# Autodesk Inventor assembly: стенка
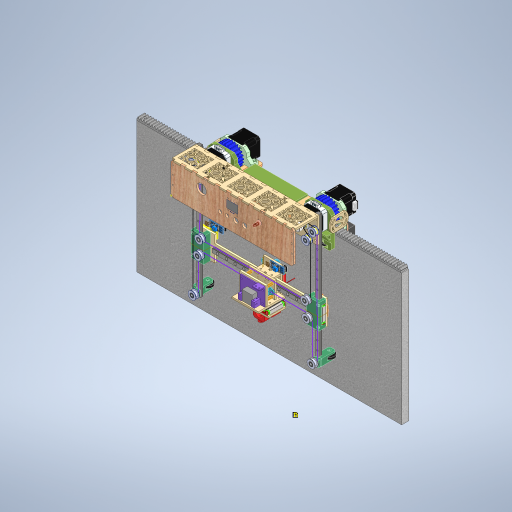
[picture p0: Inventor's stored thumbnail of the model, 512x512]
Saved by Autodesk Inventor 2024 (Build 280153000, 153)
## iProperties
Created: 2025-12-01
Part Number: стенка
Document SubType Name: Assembly
Designer: DELL
Author: DELL
## Documents named in this file (10)
- C:\Users\ejenie\reposGits\VSOSH25-26\models\poligon\poligon.iam
- C:\Users\ejenie\reposGits\VSOSH25-26\models\import\m2_20.ipt
- C:\Users\ejenie\reposGits\VSOSH25-26\models\actuator\actuator_actual\actuator.iam
- C:\Users\ejenie\reposGits\VSOSH25-26\models\plotter\plotter_actual\plotter_new.iam
- C:\Users\ejenie\reposGits\VSOSH25-26\models\actuator\actuator_mir_actual\actuator_MIR.iam
- C:\Users\ejenie\reposGits\VSOSH25-26\models\poligon\стена_полигона.ipt
- C:\Users\ejenie\reposGits\VSOSH25-26\models\plotter\plotter_actual\Сборка_электр.iam
- C:\Users\ejenie\reposGits\VSOSH25-26\models\plotter\plotter_actual\ребро_электроника.ipt
- C:\Users\ejenie\reposGits\VSOSH25-26\models\plotter\plotter_actual\плата.ipt
- C:\Users\ejenie\reposGits\VSOSH25-26\models\plotter\plotter_actual\krepezh.ipt
## Components (12 placed, 9 different names)
1. m2_20:1 — Совмещение:5, Совмещение:26, Заподлицо:2
2. m2_20:2 — Совмещение:3, Совмещение:23, Совмещение:24
3. m2_20:3 — Совмещение:3, Совмещение:5, Совмещение:25
4. actuator:1 [sub-assembly] — Совмещение:28, Заподлицо:3, Совмещение:29, Совмещение:30, Совмещение:31, Совмещение:41, Совмещение:46, Совмещение:47
5. plotter_new:1 [sub-assembly] — Совмещение:29, Совмещение:30, Совмещение:31, Совмещение:32
6. actuator_MIR:1 [sub-assembly] — Совмещение:27, Заподлицо:4, Совмещение:32, Совмещение:39, Совмещение:40, Совмещение:45, Совмещение:48, Совмещение:49
7. стена_полигона:1 — Совмещение:23, Совмещение:24, Совмещение:25, Совмещение:26, Заподлицо:2, Совмещение:27, Совмещение:28, Заподлицо:3, Заподлицо:4
8. Сборка_электр:1 [sub-assembly] — Совмещение:39, Совмещение:40, Совмещение:41, Совмещение:42, Совмещение:43, Заподлицо:5
9. ребро_электроника:1 — Совмещение:42, Совмещение:43, Заподлицо:5, Совмещение:44
10. плата:1 — Совмещение:44, Совмещение:45
11. krepezh:1 — Совмещение:46, Совмещение:47
12. krepezh:2 — Совмещение:48, Совмещение:49
## Relationships (27: Mate 23, Flush 4)
- Совмещение:3 [Mate]: m2_20:2 ↔ m2_20:3
- Совмещение:5 [Mate]: m2_20:1 ↔ m2_20:3
- Совмещение:23 [Mate]: m2_20:2 ↔ стена_полигона:1
- Совмещение:24 [Mate]: m2_20:2 ↔ стена_полигона:1
- Совмещение:25 [Mate]: m2_20:3 ↔ стена_полигона:1
- Совмещение:26 [Mate]: m2_20:1 ↔ стена_полигона:1
- Заподлицо:2 [Flush]: m2_20:1 ↔ стена_полигона:1
- Совмещение:27 [Mate] (2 mm): actuator_MIR:1 ↔ стена_полигона:1
- Совмещение:28 [Mate] (1.1 mm): actuator:1 ↔ стена_полигона:1
- Заподлицо:3 [Flush] (-50 mm): actuator:1 ↔ стена_полигона:1
- Заподлицо:4 [Flush] (-50 mm): actuator_MIR:1 ↔ стена_полигона:1
- Совмещение:29 [Mate]: actuator:1 ↔ plotter_new:1
- Совмещение:30 [Mate]: actuator:1 ↔ plotter_new:1
- Совмещение:31 [Mate]: actuator:1 ↔ plotter_new:1
- Совмещение:32 [Mate]: plotter_new:1 ↔ actuator_MIR:1
- Совмещение:39 [Mate]: actuator_MIR:1 ↔ Сборка_электр:1
- Совмещение:40 [Mate]: actuator_MIR:1 ↔ Сборка_электр:1
- Совмещение:41 [Mate]: actuator:1 ↔ Сборка_электр:1
- Совмещение:42 [Mate]: Сборка_электр:1 ↔ ребро_электроника:1
- Совмещение:43 [Mate]: Сборка_электр:1 ↔ ребро_электроника:1
- Заподлицо:5 [Flush]: Сборка_электр:1 ↔ ребро_электроника:1
- Совмещение:44 [Mate] (4 mm): ребро_электроника:1 ↔ плата:1
- Совмещение:45 [Mate] (3 mm): actuator_MIR:1 ↔ плата:1
- Совмещение:46 [Mate]: actuator:1 ↔ krepezh:1
- Совмещение:47 [Mate]: actuator:1 ↔ krepezh:1
- Совмещение:48 [Mate]: actuator_MIR:1 ↔ krepezh:2
- Совмещение:49 [Mate]: actuator_MIR:1 ↔ krepezh:2
